# Autodesk Inventor assembly: Assembly
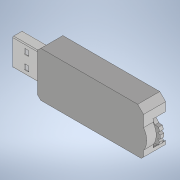
[picture p0: Inventor's stored thumbnail of the model, 180x180]
Saved by Autodesk Inventor 2020 (Build 240168000, 168)
## iProperties
Created: 2022-08-09
Part Number: Assembly
Document SubType Name: Assembly
Designer: NoName
Author: NoName
## Documents named in this file (5)
- C:\GitHub\Keyholder2\V2\3d_models\Assembly.iam
- C:\GitHub\Keyholder2\V2\3d_models\New_case.ipt
- C:\GitHub\Keyholder2\V2\3d_models\PCB.iam
- C:\GitHub\Keyholder2\V2\3d_models\Components\Battery.ipt
- C:\GitHub\Keyholder2\V2\3d_models\Components\Display_1.3_inch.ipt
## Components (4 placed, 4 different names)
1. New_case:1 — Совмещение:1, Совмещение:2, Совмещение:3, Совмещение:6, Совмещение:7, Совмещение:8
2. PCB:1 [sub-assembly] — Совмещение:1, Совмещение:2, Совмещение:3, Совмещение:4
3. Battery:1 — Совмещение:4
4. Display_1.3_inch:1 — Совмещение:6, Совмещение:7, Совмещение:8
## Relationships (7: Mate 7)
- Совмещение:1 [Mate] (0.1 mm): New_case:1 ↔ PCB:1
- Совмещение:2 [Mate] (0.2 mm): New_case:1 ↔ PCB:1
- Совмещение:3 [Mate] (0.2 mm): New_case:1 ↔ PCB:1
- Совмещение:4 [Mate] (0.1 mm): PCB:1 ↔ Battery:1
- Совмещение:6 [Mate] (0.2 mm): New_case:1 ↔ Display_1.3_inch:1
- Совмещение:7 [Mate]: New_case:1 ↔ Display_1.3_inch:1
- Совмещение:8 [Mate] (0.2 mm): New_case:1 ↔ Display_1.3_inch:1
